# Autodesk Inventor assembly: Samantha_Module
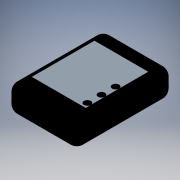
[picture p0: Inventor's stored thumbnail of the model, 180x180]
Saved by Autodesk Inventor 2017.1 (Build 211199000, 199)
## iProperties
Category: Module
Company: Autodesk Inc.
Created: 2014-11-20
Part Number: Samantha_Module
Document SubType Name: Assembly
Designer: Samantha
Vendor: US FIRST
Author: Autodesk Inc.
## Documents named in this file (3)
- D:\FIRST\FTC KOP 2017\FTC 2017 KOP\Tetrix\Miscellaneous\Samantha_Module.iam
- D:\FIRST\FTC KOP 2017\FTC 2017 KOP\Tetrix\Miscellaneous\Samantha_Case_Top.ipt
- D:\FIRST\FTC KOP 2017\FTC 2017 KOP\Tetrix\Miscellaneous\Samantha_Case_Bottom.ipt
## Components (2 placed, 2 different names)
1. Samantha_Case_Top — Mate:1, Mate:2, Mate:3
2. Samantha_Case_Bottom — Mate:1, Mate:2, Mate:3
## Relationships (3: Mate 3)
- Mate:1: Samantha_Case_Top ↔ Samantha_Case_Bottom
- Mate:2: Samantha_Case_Top ↔ Samantha_Case_Bottom
- Mate:3: Samantha_Case_Top ↔ Samantha_Case_Bottom
